# Autodesk Inventor assembly: ASY NDM 11.040 рама 3 вертикал угол
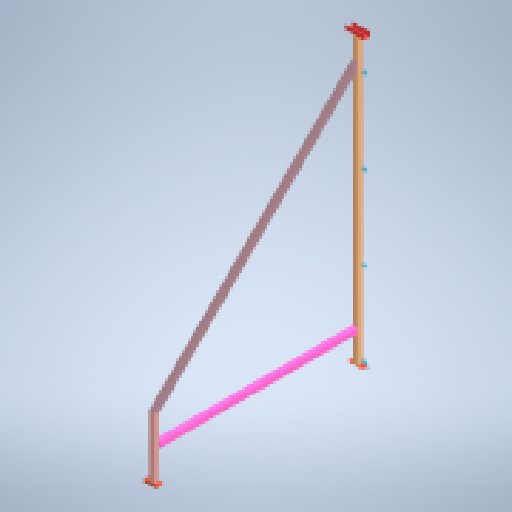
[picture p0: Inventor's stored thumbnail of the model, 512x512]
Saved by Autodesk Inventor 2025 (Build 290162010, 162A)
## iProperties
Created: 2024-06-21
Part Number: ASY NDM 11.040 рама 3 вертикал угол
Document SubType Name: Assembly
Designer: admin
_SolveAssemblyDoc: Frame Generator Solve Assembly
_Version: 25.0.0
Author: admin
## Documents named in this file (6)
- C:\Users\admin\YandexDisk-badmisterfox\домашниий пк\Inventor\Nadyim\CAD\Перегородка\ASY NDM 11.040 рама 3 вертикал угол.iam
- C:\Users\admin\YandexDisk-badmisterfox\домашниий пк\Inventor\Nadyim\CAD\Перегородка\NDM 11.041 рама 3 вертикал угол.ipt
- C:\Users\admin\YandexDisk-badmisterfox\домашниий пк\Inventor\Nadyim\CAD\Перегородка\ASY NDM 11.040 рама 3 вертикал угол\Frame\Frame 1718954205588.iam
- C:\Users\admin\YandexDisk-badmisterfox\домашниий пк\Inventor\Nadyim\CAD\кронштейн\NDM 4.0.9 кронштейн связь 9.ipt
- C:\Users\admin\YandexDisk-badmisterfox\домашниий пк\Inventor\Nadyim\CAD\кронштейн\NDM 11.027 кронштейн 27.ipt
- C:\Users\admin\YandexDisk-badmisterfox\домашниий пк\Inventor\Nadyim\CAD\кронштейн\NDM 11.028 кронштейн 28.ipt
## Components (9 placed, 5 different names)
1. NDM 11.041 рама 3 вертикал угол:1
2. Frame 1718954205588:1 [sub-assembly] — Rigid:1, Rigid:2, Rigid:3, Rigid:4
3. NDM 4.0.9 кронштейн связь 9:1 — Rigid:1
4. NDM 4.0.9 кронштейн связь 9:2 — Rigid:2
5. NDM 11.027 кронштейн 27:1 — Rigid:3
6. NDM 11.028 кронштейн 28:1 — Rigid:4
7. NDM 11.028 кронштейн 28:2
8. NDM 11.028 кронштейн 28:3
9. NDM 11.028 кронштейн 28:4
## Component patterns: (4 elements, first: NDM 11.028 кронштейн 28:1)
## Relationships (4: WeldJoint 4)
- Rigid:1 [WeldJoint]: Frame 1718954205588:1 ↔ NDM 4.0.9 кронштейн связь 9:1
- Rigid:2 [WeldJoint]: Frame 1718954205588:1 ↔ NDM 4.0.9 кронштейн связь 9:2
- Rigid:3 [WeldJoint]: Frame 1718954205588:1 ↔ NDM 11.027 кронштейн 27:1
- Rigid:4 [WeldJoint]: Frame 1718954205588:1 ↔ NDM 11.028 кронштейн 28:1
